# Autodesk Inventor assembly: EDM Wire layout
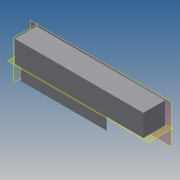
[picture p0: Inventor's stored thumbnail of the model, 180x180]
Saved by Autodesk Inventor 2015 (Build 190159000, 159)
## iProperties
Created: 2015-08-11
Part Number: EDM Wire layout
Document SubType Name: Assembly
Designer: jdyne
Author: jdyne
## Documents named in this file (3)
- D:\Documents\Inventor\Microwave Transmission line\Graphite absorber\EDM Wire layout.iam
- D:\Documents\Inventor\Microwave Transmission line\Graphite absorber\Ferrite Absorber.ipt
- D:\Documents\Inventor\Microwave Transmission line\Graphite absorber\Wedge.ipt
## Components (3 placed, 2 different names)
1. Ferrite Absorber:1 — Mate:2, Flush:1, Flush:2, Flush:3, Mate:3, Flush:4, Mate:4, Mate:5, Mate:6
2. Wedge:1 — Mate:2, Flush:1, Flush:2
3. Wedge:2 — Flush:3, Mate:3, Flush:4
## Relationships (9: Mate 5, Flush 4)
- Mate:2: Ferrite Absorber:1 ↔ Wedge:1
- Flush:1 (-2 mm): Ferrite Absorber:1 ↔ Wedge:1
- Flush:2 (-5 mm): Ferrite Absorber:1 ↔ Wedge:1
- Flush:3 (-5 mm): Ferrite Absorber:1 ↔ Wedge:2
- Mate:3: Ferrite Absorber:1 ↔ Wedge:2
- Flush:4 (-2 mm): Ferrite Absorber:1 ↔ Wedge:2
- Mate:4: Ferrite Absorber:1
- Mate:5: Ferrite Absorber:1
- Mate:6: Ferrite Absorber:1
